# Autodesk Inventor assembly: Sorting Full Mechanism
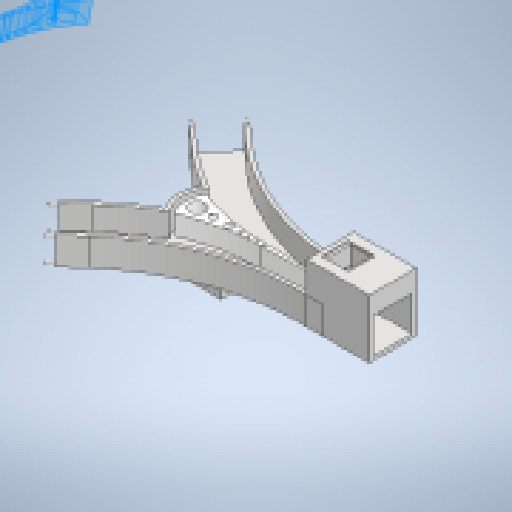
[picture p0: Inventor's stored thumbnail of the model, 512x512]
Saved by Autodesk Inventor 2025.3 (Build 293356000, 356)
## iProperties
Created: 2026-04-18
Part Number: Sorting Full Mechanism
Document SubType Name: Assembly
Designer: kamal
Author: kamal
## Documents named in this file (8)
- C:\Users\kamal\OneDrive\Desktop\Personal\semester 4\Basics of Mechatronics\Full Assembly\Sorting Full Mechanism.iam
- C:\Users\kamal\OneDrive\Desktop\Personal\semester 4\Basics of Mechatronics\Full Assembly\Sorting_Body_Final.ipt
- C:\Users\kamal\OneDrive\Desktop\Personal\semester 4\Basics of Mechatronics\Full Assembly\servo_holder_V2.ipt
- C:\Users\kamal\OneDrive\Desktop\Personal\semester 4\Basics of Mechatronics\Full Assembly\SG90_Model_A.ipt
- C:\Users\kamal\OneDrive\Desktop\Personal\semester 4\Basics of Mechatronics\Full Assembly\SG90_Arm_Original.ipt
- C:\Users\kamal\OneDrive\Desktop\Personal\semester 4\Basics of Mechatronics\Full Assembly\Servo_Shaft_V2.ipt
- C:\Users\kamal\OneDrive\Desktop\Personal\semester 4\Basics of Mechatronics\Full Assembly\mover.ipt
- C:\Users\kamal\OneDrive\Desktop\Personal\semester 4\Basics of Mechatronics\Full Assembly\color sensor holder.ipt
## Components (7 placed, 7 different names)
1. Sorting_Body_Final:1 — Insert:4, Insert:5, Mate:4, Mate:5
2. servo_holder_V2:1 — Insert:1, Insert:2, Insert:4, Insert:5
3. SG90_Arm_Original:1 — Insert:3, Mate:1, Mate:2
4. SG90_Model_A:1 — Insert:1, Insert:2, Insert:3
5. Servo_Shaft_V2:1 — Mate:1, Mate:2, Insert:6, Mate:3
6. mover:1 — Insert:6, Mate:3
7. color sensor holder:1 — Mate:4, Mate:5
## Relationships (11: Insert 6, Mate 5)
- Insert:1: servo_holder_V2:1 ↔ SG90_Model_A:1
- Insert:2: servo_holder_V2:1 ↔ SG90_Model_A:1
- Insert:3: SG90_Arm_Original:1 ↔ SG90_Model_A:1
- Mate:1: SG90_Arm_Original:1 ↔ Servo_Shaft_V2:1
- Mate:2: SG90_Arm_Original:1 ↔ Servo_Shaft_V2:1
- Insert:4: Sorting_Body_Final:1 ↔ servo_holder_V2:1
- Insert:5: Sorting_Body_Final:1 ↔ servo_holder_V2:1
- Insert:6: Servo_Shaft_V2:1 ↔ mover:1
- Mate:3: Servo_Shaft_V2:1 ↔ mover:1
- Mate:4: Sorting_Body_Final:1 ↔ color sensor holder:1
- Mate:5: Sorting_Body_Final:1 ↔ color sensor holder:1
